# Autodesk Inventor assembly: 95646c01
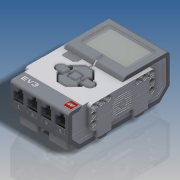
[picture p0: Inventor's stored thumbnail of the model, 180x180]
Saved by Autodesk Inventor 2016 SP2 (Build 200236200, 236)
## iProperties
Created: 2015-08-20
Part Number: 95646c01
Document SubType Name: Assembly
Designer: D. Kohfeld
Mass: 106.628 g
Surface Area: 1531.99 cm^2
Volume: 98.023 cm^3
Density: 1.08778 g/cm^3
Author: D. Kohfeld
## Documents named in this file (21)
- A:\LEGO Pieces\EV3\95646c01.iam
- A:\LEGO Pieces\EV3\99141p01-White.ipt
- A:\LEGO Pieces\EV3\11026-TransClear.ipt
- A:\LEGO Pieces\EV3\11030-LtBluishGray.ipt
- A:\LEGO Pieces\EV3\11036-LCD.ipt
- A:\LEGO Pieces\EV3\99145-LtBluishGray.ipt
- A:\LEGO Pieces\EV3\99146-LtBluishGray.ipt
- A:\LEGO Pieces\EV3\99147-LtBluishGray.ipt
- A:\LEGO Pieces\EV3\99148p01-TransClear.ipt
- A:\LEGO Pieces\EV3\99141s01-LtBluishGray.ipt
- A:\LEGO Pieces\EV3\95656.iam
- A:\LEGO Pieces\EV3\11025-White.ipt
- A:\LEGO Pieces\EV3\11025s02-LtBluishGray.ipt
- A:\LEGO Pieces\EV3\11032-Black.ipt
- A:\LEGO Pieces\EV3\11033-Black.ipt
- A:\LEGO Pieces\#data.ipt
- A:\LEGO Pieces\EV3\11034-Black.ipt
- A:\LEGO Pieces\EV3\11035-LtBluishGray.ipt
- A:\LEGO Pieces\EV3\54732b-LtBluishGray.ipt
- A:\LEGO Pieces\EV3\97622-PCB.ipt
- A:\LEGO Pieces\EV3\99143-LtBluishGray.ipt
## Components (24 placed, 19 different names)
1. 99141p01-White:1 — Mate:1, Mate:2, Flush:1, Mate:3, Flush:2, Flush:4, Flush:5, Flush:7, Flush:8, Flush:11, Flush:12, Flush:13, Flush:14, Mate:16, Mate:10, Flush:17, Flush:18, Mate:17, Flush:20, Flush:21, Mate:20, Mate:21, Mate:26, Mate:27, Mate:28, Flush:28, Mate:40, Flush:29
2. 11026-TransClear:1 — Flush:1, Mate:3, Flush:2, Flush:3, Mate:4, Mate:5, Mate:6, Flush:6, Mate:7, Mate:8, Mate:9, Flush:9, Flush:10, Mate:39
3. 11030-LtBluishGray:1 — Mate:1, Mate:2
4. 11036-LCD:1 — Flush:13
5. 99145-LtBluishGray:1 — Flush:6, Mate:9, Flush:7
6. 99145-LtBluishGray:2 — Mate:7, Mate:8, Flush:8
7. 99146-LtBluishGray:1 — Flush:9, Flush:10, Flush:11
8. 99147-LtBluishGray:1 — Mate:4, Mate:6, Flush:4
9. 99147-LtBluishGray:2 — Flush:3, Mate:5, Flush:5
10. 99148p01-TransClear:1 — Flush:12, Mate:11, Flush:16
11. 99141s01-LtBluishGray:1 — Flush:14, Mate:16, Mate:10, Mate:11, Flush:16, Mate:23, Mate:24, Mate:25, Flush:23, Mate:30, Mate:35, Mate:36, Mate:37, Mate:38, Flush:24, Flush:25, Flush:26, Flush:27
12. 95656:1 [sub-assembly] — Flush:21, Flush:22, Mate:19
13. 11025-White:1 — Flush:17, Flush:18, Mate:17, Flush:19, Mate:18, Mate:19, Mate:22, Mate:41, Flush:30
14. 11025s02-LtBluishGray:1 — Flush:19, Flush:20, Mate:18, Flush:22, Mate:29, Mate:31, Mate:32, Mate:33, Mate:34
15. 11032-Black:1 — Mate:20, Mate:21, Mate:22
16. 11033-Black:1 — Mate:23, Mate:24, Mate:25
17. 11034-Black:1 — Mate:26, Mate:27, Mate:28
18. 11035-LtBluishGray:1 — Flush:23, Mate:29, Mate:30
19. 54732b-LtBluishGray:1 — Mate:31, Mate:35, Flush:24
20. 54732b-LtBluishGray:2 — Mate:32, Mate:36, Flush:25
21. 54732b-LtBluishGray:3 — Mate:33, Mate:37, Flush:26
22. 54732b-LtBluishGray:4 — Mate:34, Mate:38, Flush:27
23. 97622-PCB:1 — Flush:28, Mate:39, Mate:40
24. 99143-LtBluishGray:1 — Flush:29, Mate:41, Flush:30
## Relationships (66: Mate 37, Flush 29)
- Mate:1: 99141p01-White:1 ↔ 11030-LtBluishGray:1
- Mate:2: 99141p01-White:1 ↔ 11030-LtBluishGray:1
- Flush:1: 99141p01-White:1 ↔ 11026-TransClear:1
- Mate:3: 99141p01-White:1 ↔ 11026-TransClear:1
- Flush:2: 99141p01-White:1 ↔ 11026-TransClear:1
- Flush:3: 11026-TransClear:1 ↔ 99147-LtBluishGray:2
- Mate:4: 11026-TransClear:1 ↔ 99147-LtBluishGray:1
- Mate:5: 11026-TransClear:1 ↔ 99147-LtBluishGray:2
- Mate:6: 11026-TransClear:1 ↔ 99147-LtBluishGray:1
- Flush:4: 99141p01-White:1 ↔ 99147-LtBluishGray:1
- Flush:5: 99141p01-White:1 ↔ 99147-LtBluishGray:2
- Flush:6: 11026-TransClear:1 ↔ 99145-LtBluishGray:1
- Mate:7: 11026-TransClear:1 ↔ 99145-LtBluishGray:2
- Mate:8: 11026-TransClear:1 ↔ 99145-LtBluishGray:2
- Mate:9: 11026-TransClear:1 ↔ 99145-LtBluishGray:1
- Flush:7: 99141p01-White:1 ↔ 99145-LtBluishGray:1
- Flush:8: 99141p01-White:1 ↔ 99145-LtBluishGray:2
- Flush:9: 11026-TransClear:1 ↔ 99146-LtBluishGray:1
- Flush:10: 11026-TransClear:1 ↔ 99146-LtBluishGray:1
- Flush:11: 99141p01-White:1 ↔ 99146-LtBluishGray:1
- Flush:12: 99141p01-White:1 ↔ 99148p01-TransClear:1
- Flush:13: 99141p01-White:1 ↔ 11036-LCD:1
- Flush:14: 99141p01-White:1 ↔ 99141s01-LtBluishGray:1
- Mate:16: 99141p01-White:1 ↔ 99141s01-LtBluishGray:1
- Mate:10: 99141p01-White:1 ↔ 99141s01-LtBluishGray:1
- Mate:11: 99148p01-TransClear:1 ↔ 99141s01-LtBluishGray:1
- Flush:16: 99148p01-TransClear:1 ↔ 99141s01-LtBluishGray:1
- Flush:17: 99141p01-White:1 ↔ 11025-White:1
- Flush:18: 99141p01-White:1 ↔ 11025-White:1
- Mate:17: 99141p01-White:1 ↔ 11025-White:1
- Flush:19: 11025-White:1 ↔ 11025s02-LtBluishGray:1
- Flush:20: 99141p01-White:1 ↔ 11025s02-LtBluishGray:1
- Mate:18: 11025-White:1 ↔ 11025s02-LtBluishGray:1
- Flush:21: 99141p01-White:1 ↔ 95656:1
- Flush:22: 95656:1 ↔ 11025s02-LtBluishGray:1
- Mate:19: 95656:1 ↔ 11025-White:1
- Mate:20: 99141p01-White:1 ↔ 11032-Black:1
- Mate:21: 99141p01-White:1 ↔ 11032-Black:1
- Mate:22: 11025-White:1 ↔ 11032-Black:1
- Mate:23 (1.6 mm): 99141s01-LtBluishGray:1 ↔ 11033-Black:1
- Mate:24: 99141s01-LtBluishGray:1 ↔ 11033-Black:1
- Mate:25: 99141s01-LtBluishGray:1 ↔ 11033-Black:1
- Mate:26: 99141p01-White:1 ↔ 11034-Black:1
- Mate:27: 99141p01-White:1 ↔ 11034-Black:1
- Mate:28: 99141p01-White:1 ↔ 11034-Black:1
- Flush:23: 99141s01-LtBluishGray:1 ↔ 11035-LtBluishGray:1
- Mate:29: 11025s02-LtBluishGray:1 ↔ 11035-LtBluishGray:1
- Mate:30: 99141s01-LtBluishGray:1 ↔ 11035-LtBluishGray:1
- Mate:31: 11025s02-LtBluishGray:1 ↔ 54732b-LtBluishGray:1
- Mate:32: 11025s02-LtBluishGray:1 ↔ 54732b-LtBluishGray:2
- Mate:33: 11025s02-LtBluishGray:1 ↔ 54732b-LtBluishGray:3
- Mate:34: 11025s02-LtBluishGray:1 ↔ 54732b-LtBluishGray:4
- Mate:35: 99141s01-LtBluishGray:1 ↔ 54732b-LtBluishGray:1
- Mate:36: 99141s01-LtBluishGray:1 ↔ 54732b-LtBluishGray:2
- Mate:37: 99141s01-LtBluishGray:1 ↔ 54732b-LtBluishGray:3
- Mate:38: 99141s01-LtBluishGray:1 ↔ 54732b-LtBluishGray:4
- Flush:24: 99141s01-LtBluishGray:1 ↔ 54732b-LtBluishGray:1
- Flush:25: 99141s01-LtBluishGray:1 ↔ 54732b-LtBluishGray:2
- Flush:26: 99141s01-LtBluishGray:1 ↔ 54732b-LtBluishGray:3
- Flush:27: 99141s01-LtBluishGray:1 ↔ 54732b-LtBluishGray:4
- Flush:28: 99141p01-White:1 ↔ 97622-PCB:1
- Mate:39: 11026-TransClear:1 ↔ 97622-PCB:1
- Mate:40: 99141p01-White:1 ↔ 97622-PCB:1
- Flush:29: 99141p01-White:1 ↔ 99143-LtBluishGray:1
- Mate:41: 11025-White:1 ↔ 99143-LtBluishGray:1
- Flush:30: 11025-White:1 ↔ 99143-LtBluishGray:1
## Named parameters: lu = 8 mm, kd = 4.8 mm, wall = 1.6 mm, lh = 9.6 mm, knobh = 1.6 mm, bd = 8 mm, rd = 3.2 mm, topthk = 1.6 mm, tubeod = 6.51371 mm, axlet = 1.6 mm, pd = 3.2 mm, gw = 0.4 mm, gh = 0.4 mm, tpd = 4.8 mm, tpcd = 5 mm, tsd = 6.2 mm, th = 5.6 mm, tsl = 0.8 mm, tpnw = 0.8 mm, tpnl = 3.4 mm, tlad = 7.2 mm
